# Autodesk Inventor assembly: 120 mm fan assembly
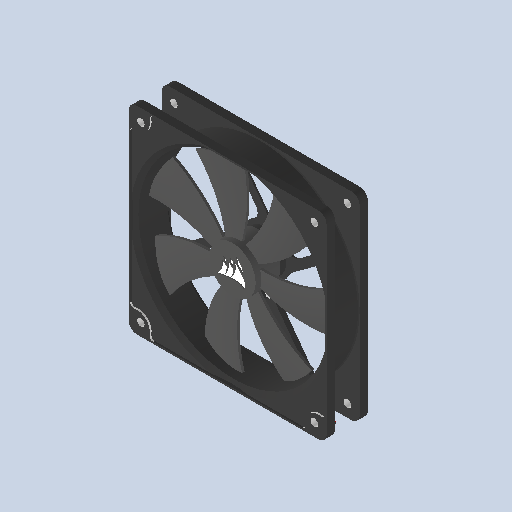
[picture p0: Inventor's stored thumbnail of the model, 512x512]
Saved by Autodesk Inventor 2022 (Build 260153000, 153)
## iProperties
Created: 2021-05-19
Part Number: 120 mm fan assembly
Document SubType Name: Assembly
Designer: 6128059
Author: 6128059
## Documents named in this file (3)
- C:\Users\sbbgi\Documents\GitHub\eatx_case\atx\resources\aio-cooler-1.snapshot.2\AIO Cooler\120 mm fan assembly.iam
- C:\Users\sbbgi\Documents\GitHub\eatx_case\atx\resources\aio-cooler-1.snapshot.2\AIO Cooler\Pc Fan 120 mm - Housing.ipt
- C:\Users\sbbgi\Documents\GitHub\eatx_case\atx\resources\aio-cooler-1.snapshot.2\AIO Cooler\Pc Fan 120 mm - fan.ipt
## Components (2 placed, 2 different names)
1. Pc Fan 120 mm - Housing:1 — Insert:1, Angle:1
2. Pc Fan 120 mm - fan:1 — Insert:1, Angle:1
## Relationships (2: Insert 1, Angle 1)
- Insert:1: Pc Fan 120 mm - Housing:1 ↔ Pc Fan 120 mm - fan:1
- Angle:1 (0 deg): Pc Fan 120 mm - Housing:1 ↔ Pc Fan 120 mm - fan:1
